# Autodesk Inventor assembly: Drive2
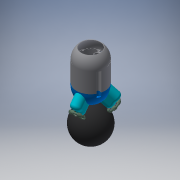
[picture p0: Inventor's stored thumbnail of the model, 180x180]
Saved by Autodesk Inventor 2018.3 (Build 223284000, 284)
## iProperties
Created: 2018-06-30
Part Number: Drive2
Material: Generisch
Document SubType Name: Assembly
Designer: JochenAlt
Author: JochenAlt
## Documents named in this file (3)
- D:\Projects\Ondine\CAD\Drive.iam
- D:\Projects\Ondine\CAD\Sphere.ipt
- D:\Projects\Ondine\CAD\DriveChain.iam
## Components (4 placed, 2 different names)
1. Sphere:1 — Passend:38, Passend:61
2. DriveChain:1 [sub-assembly] — Passend:60, Passend:61, Passend:62, Passend:63, Passend:64
3. DriveChain:2 [sub-assembly] — Passend:62, Passend:63, Passend:65
4. DriveChain:3 [sub-assembly] — Passend:64, Passend:65
## Relationships (7: Mate 7)
- Passend:38 [Mate]: Sphere:1
- Passend:60 [Mate]: DriveChain:1
- Passend:61 [Mate] (89 mm): Sphere:1 ↔ DriveChain:1
- Passend:62 [Mate]: DriveChain:1 ↔ DriveChain:2
- Passend:63 [Mate]: DriveChain:1 ↔ DriveChain:2
- Passend:64 [Mate]: DriveChain:1 ↔ DriveChain:3
- Passend:65 [Mate]: DriveChain:2 ↔ DriveChain:3
